# Autodesk Inventor assembly: rev4
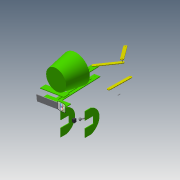
[picture p0: Inventor's stored thumbnail of the model, 180x180]
Saved by Autodesk Inventor 2015 (Build 190159000, 159)
## iProperties
Created: 2014-07-15
Part Number: rev4
Document SubType Name: Assembly
Designer: shohei
Author: shohei
## Documents named in this file (13)
- C:\Users\shohei\Documents\Inventor\FufuPounder\rev4.iam
- C:\Users\shohei\Documents\Inventor\FufuPounder\Part1.ipt
- C:\Users\shohei\Documents\Inventor\FufuPounder\Part2.ipt
- C:\Users\shohei\Documents\Inventor\FufuPounder\Part4.ipt
- C:\Users\shohei\Documents\Inventor\FufuPounder\baseboard.ipt
- C:\Users\shohei\Documents\Inventor\FufuPounder\shaft2.ipt
- C:\Users\shohei\Documents\Inventor\FufuPounder\shaft3.ipt
- C:\Users\shohei\Documents\Inventor\FufuPounder\mallet_aseembly.iam
- C:\Users\shohei\Documents\Inventor\CNC_Plasma_Cutter\main\42BYGHM809.ipt
- C:\Users\shohei\Documents\Inventor\FufuPounder\mortar2.ipt
- C:\Users\shohei\Documents\Inventor\FufuPounder\beam.ipt
- C:\Users\shohei\Documents\Inventor\FufuPounder\small_lever.ipt
- C:\Users\shohei\Documents\Inventor\FufuPounder\shaft.ipt
## Components (15 placed, 12 different names)
1. Part1:1 — Slider:1, Rigid:2, Mate:2, Flush:12, Flush:14
2. Part1:2 — Flush:15
3. Part4:1 — Rotational:1, Rotational:2
4. Part4:2
5. baseboard:1 — Mate:2, Flush:12, Flush:14, Flush:15
6. shaft2:1 — Slider:1, Cylindrical:26
7. shaft3:1 — Rotational:2, Rotational:3
8. mallet_aseembly:1 [sub-assembly] — Cylindrical:26
9. Part2:5 — Rigid:2, Rotational:1
10. 42BYGHM809:1
11. mortar2:1
12. beam:1
13. beam:2
14. small_lever:2 — Rotational:3
15. shaft:1
## Relationships (10: RevoluteJoint 3, Flush 3, TranslationJoint 1, WeldJoint 1, CylindricalJoint 1, Mate 1)
- Slider:1 [TranslationJoint]: Part1:1 ↔ shaft2:1
- Rigid:2 [WeldJoint]: Part1:1 ↔ Part2:5
- Cylindrical:26: shaft2:1 ↔ mallet_aseembly:1
- Rotational:1 [RevoluteJoint]: Part4:1 ↔ Part2:5
- Rotational:2 [RevoluteJoint]: Part4:1 ↔ shaft3:1
- Rotational:3 [RevoluteJoint]: shaft3:1 ↔ small_lever:2
- Mate:2: Part1:1 ↔ baseboard:1
- Flush:12: Part1:1 ↔ baseboard:1
- Flush:14: Part1:1 ↔ baseboard:1
- Flush:15: Part1:2 ↔ baseboard:1
